# Autodesk Inventor assembly: Tracker
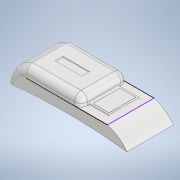
[picture p0: Inventor's stored thumbnail of the model, 180x180]
Saved by Autodesk Inventor 2020 (Build 240168000, 168)
## iProperties
Created: 2019-07-11
Part Number: Tracker
Document SubType Name: Assembly
Designer: tyrre
Author: tyrre
## Documents named in this file (6)
- C:\Users\tyrre\Downloads\moteino-pcb-trace-antenna-1.snapshot.4\Tracker.iam
- C:\Users\tyrre\OneDrive\Desktop\University - Ryan\Work\Work - 2019\Inventor Files\Battery.ipt
- C:\Users\tyrre\OneDrive\Desktop\University - Ryan\Work\Work - 2019\Inventor Files\GPS.ipt
- C:\Users\tyrre\OneDrive\Desktop\University - Ryan\Work\Work - 2019\Inventor Files\MoteinoPCB.ipt
- C:\Users\tyrre\OneDrive\Desktop\University - Ryan\Work\Work - 2019\Inventor Files\Case - Bottom.ipt
- C:\Users\tyrre\OneDrive\Desktop\University - Ryan\Work\Work - 2019\Inventor Files\Case - Top.ipt
## Components (5 placed, 5 different names)
1. Battery:1 — Mate:1, Flush:2, Flush:3, Flush:5, Mate:3, Mate:4, Mate:5
2. GPS:1 — Mate:2, Flush:4, Flush:5, Mate:6, Mate:7
3. MoteinoPCB:1 — Mate:1, Flush:2, Flush:3, Mate:2, Flush:4
4. Case - Bottom:1 — Mate:3, Mate:4, Mate:5
5. Case - Top:1 — Mate:6, Mate:7
## Relationships (11: Mate 7, Flush 4)
- Mate:1: Battery:1 ↔ MoteinoPCB:1
- Flush:2 (1.193 mm): Battery:1 ↔ MoteinoPCB:1
- Flush:3: Battery:1 ↔ MoteinoPCB:1
- Mate:2: GPS:1 ↔ MoteinoPCB:1
- Flush:4: GPS:1 ↔ MoteinoPCB:1
- Flush:5 (8.75 mm): Battery:1 ↔ GPS:1
- Mate:3: Battery:1 ↔ Case - Bottom:1
- Mate:4: Battery:1 ↔ Case - Bottom:1
- Mate:5: Battery:1 ↔ Case - Bottom:1
- Mate:6: GPS:1 ↔ Case - Top:1
- Mate:7: GPS:1 ↔ Case - Top:1
